# Autodesk Inventor assembly: HERRAMIENTA
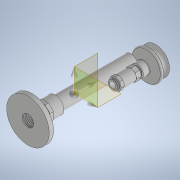
[picture p0: Inventor's stored thumbnail of the model, 180x180]
Saved by Autodesk Inventor 2022 (Build 260153000, 153)
## iProperties
Created: 2022-09-01
Part Number: HERRAMIENTA
Document SubType Name: Assembly
Designer: Usuario
Mass: 160 g
Surface Area: 461.668 cm^2
Volume: 76.1228 cm^3
Author: Usuario
## Documents named in this file (5)
- C:\Users\Usuario\Documents\Cosas de Sebastian\Robotica\PROYECTO\CAD\HERRAMIENTA\HERRAMIENTA.iam
- C:\Users\Usuario\Documents\Cosas de Sebastian\Robotica\PROYECTO\CAD\HERRAMIENTA\ACOPLE.ipt
- C:\Users\Usuario\Documents\Cosas de Sebastian\Robotica\PROYECTO\CAD\HERRAMIENTA\FLANCHE.ipt
- C:\Users\Usuario\Documents\Cosas de Sebastian\Robotica\PROYECTO\CAD\HERRAMIENTA\TUBO.ipt
- C:\Users\Usuario\Documents\Cosas de Sebastian\Robotica\PROYECTO\CAD\HERRAMIENTA\ENSAMBLAJE_VENTOSA_1.iam
## Components (4 placed, 4 different names)
1. ACOPLE:1 — Coincidencia:1, Insertar:1, Coincidencia:3
2. FLANCHE:1 — Coincidencia:1, Coincidencia:2, Nivelación:1, Coincidencia:3
3. TUBO:1 — Insertar:1, Tangente:1, Tangente:2, Nivelación:2
4. ENSAMBLAJE_VENTOSA_1:1 [sub-assembly] — Tangente:1, Tangente:2, Nivelación:2
## Relationships (8: Mate 3, Flush 2, Tangent 2, Insert 1)
- Coincidencia:1 [Mate]: ACOPLE:1 ↔ FLANCHE:1
- Insertar:1: ACOPLE:1 ↔ TUBO:1
- Coincidencia:2 [Mate]: FLANCHE:1
- Nivelación:1 [Flush]: FLANCHE:1
- Coincidencia:3 [Mate]: ACOPLE:1 ↔ FLANCHE:1
- Tangente:1: TUBO:1 ↔ ENSAMBLAJE_VENTOSA_1:1
- Tangente:2: TUBO:1 ↔ ENSAMBLAJE_VENTOSA_1:1
- Nivelación:2 [Flush]: TUBO:1 ↔ ENSAMBLAJE_VENTOSA_1:1
